# Autodesk Inventor assembly: ArmEncoderBoardCorrectedFootprint
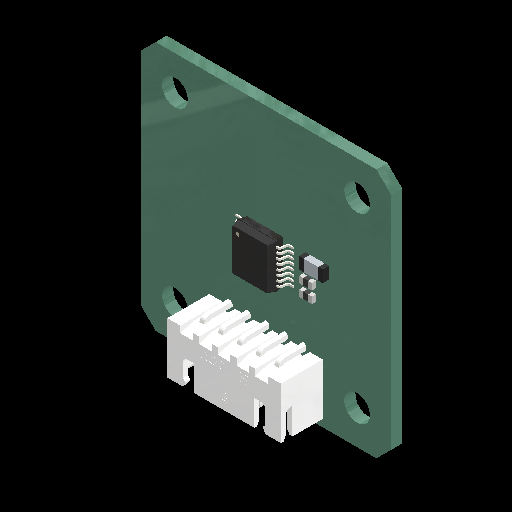
[picture p0: Inventor's stored thumbnail of the model, 512x512]
Saved by Autodesk Inventor 2025.2 (Build 292293000, 293)
## iProperties
Company: Kicad
Created: 2026-02-04
Part Number: ArmEncoderBoardCorrectedFootprint
Description: KiCad electronic assembly
Document SubType Name: Assembly
Designer: valer
Authority: Unknown
Sending System: KiCad to STEP converter
Preprocessor: Open CASCADE STEP processor 7.8
Title: ArmEncoderBoardCorrectedFootprint.step
Author: Pcbnew
## Documents named in this file (6)
- C:\Users\valer\Desktop\str1ker\cad\external\ArmEncoder\ArmEncoderBoardCorrectedFootprint.iam
- C:\Users\valer\Desktop\str1ker\cad\external\ArmEncoder\885342208002.iam
- C:\Users\valer\Desktop\str1ker\cad\external\ArmEncoder\CR0603-FX-4701ELF.ipt
- C:\Users\valer\Desktop\str1ker\cad\external\ArmEncoder\SSOP-16_5.3x6.2mm_P0.65mm.ipt
- C:\Users\valer\Desktop\str1ker\cad\external\ArmEncoder\ArmEncoderBoard_PCB.ipt
- C:\Users\valer\Desktop\str1ker\cad\external\ArmEncoder\WHITE JST XH 5 PIN CONNECTOR - P 2.54mm - ANGLED.ipt
## Components (6 placed, 6 different names)
1. 4 [sub-assembly]
2. 5
3. 6 — Flush:1
4. 8
5. 9 — Mate:1, Mate:2, Flush:2
6. WHITE JST XH 5 PIN CONNECTOR - P 2.54mm - ANGLED:1 — Mate:1, Mate:2, Flush:1, Flush:2
## Relationships (4: Mate 2, Flush 2)
- Mate:1: 9 ↔ WHITE JST XH 5 PIN CONNECTOR - P 2.54mm - ANGLED:1
- Mate:2: 9 ↔ WHITE JST XH 5 PIN CONNECTOR - P 2.54mm - ANGLED:1
- Flush:1: 6 ↔ WHITE JST XH 5 PIN CONNECTOR - P 2.54mm - ANGLED:1
- Flush:2 (1 mm): 9 ↔ WHITE JST XH 5 PIN CONNECTOR - P 2.54mm - ANGLED:1
